# Autodesk Inventor assembly: Baugruppe_Christian_Test
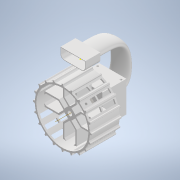
[picture p0: Inventor's stored thumbnail of the model, 180x180]
Saved by Autodesk Inventor 2021 (Build 250183000, 183)
## iProperties
Created: 2021-01-04
Part Number: Baugruppe_Christian_Test
Document SubType Name: Assembly
Designer: Ctroi
Mass: 279.93 g
Surface Area: 1178.31 cm^2
Volume: 279.93 cm^3
Density: 1 g/cm^3
Author: Ctroi
## Documents named in this file (6)
- G:\Roverprojekt\Github Projekt\Rover\Baugruppe_Christian_Test.iam
- G:\Roverprojekt\Github Projekt\Rover\Motorhalterung_v2.ipt
- G:\Roverprojekt\Github Projekt\Rover\Steppermotor.ipt
- G:\Roverprojekt\Github Projekt\Rover\Reifen_v2.ipt
- G:\Roverprojekt\Github Projekt\Rover\Verbindung_Motor_Servo.ipt
- G:\Roverprojekt\Github Projekt\Rover\Motorhalterung_Klemme.ipt
## Components (5 placed, 5 different names)
1. Motorhalterung_v2:1 — Passend:1
2. Reifen_v2:1 — Einfügen:1
3. Verbindung_Motor_Servo:1
4. Steppermotor:1 — Einfügen:1
5. Motorhalterung_Klemme:1 — Passend:1
## Relationships (2: Insert 1, Mate 1)
- Einfügen:1 [Insert] (-15 mm): Reifen_v2:1 ↔ Steppermotor:1
- Passend:1 [Mate]: Motorhalterung_v2:1 ↔ Motorhalterung_Klemme:1
